# Autodesk Inventor assembly: Pick_&_Place_Nozzle_Assembly
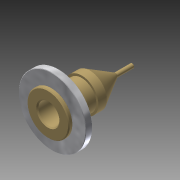
[picture p0: Inventor's stored thumbnail of the model, 180x180]
Saved by Autodesk Inventor 2015 (Build 190159000, 159)
## iProperties
Created: 2015-01-06
Part Number: Pick_&_Place_Nozzle_Assembly
Document SubType Name: Assembly
Designer: ice
Author: ice
## Documents named in this file (3)
- C:\Users\ice\Documents\GitHub\PnP-Magnetic-Tool-Tip\Inventor\Assembly_Nozzle_#2.iam
- C:\Users\ice\Documents\GitHub\PnP-Magnetic-Tool-Tip\Inventor\Nozzle#2.ipt
- C:\Users\ice\Documents\GitHub\PnP-Magnetic-Tool-Tip\Inventor\M8_Ring.ipt
## Components (2 placed, 2 different names)
1. Nozzle#2:1 — Mate:1, Mate:2, Mate:3, Flush:1
2. M8_Ring:1 — Mate:1, Mate:2
## Relationships (4: Mate 3, Flush 1)
- Mate:1: Nozzle#2:1 ↔ M8_Ring:1
- Mate:2: Nozzle#2:1 ↔ M8_Ring:1
- Mate:3: Nozzle#2:1
- Flush:1: Nozzle#2:1
